# Autodesk Inventor assembly: Coluna_Suspensao_3-Cabos_Modelo3
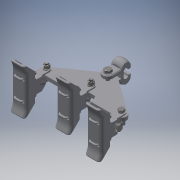
[picture p0: Inventor's stored thumbnail of the model, 180x180]
Saved by Autodesk Inventor 2018 (Build 220112000, 112)
## iProperties
Created: 2021-08-02
Part Number: Coluna_Suspensao_3-Cabos_Modelo3
Document SubType Name: Assembly
Designer: L08619
Author: L08619
## Documents named in this file (4)
- C:\Users\l08619\Documents\Projetos\TAESA\Modelo 3D - Tensionadores e Suspensão\Suporte de Suspenção\Coluna_Suspensao_3-Cabos_Modelo3.iam
- C:\Users\l08619\Documents\Projetos\TAESA\Modelo 3D - Tensionadores e Suspensão\Suporte de Suspenção\Corpo_Suporte_3_Cabos_Modelo3.ipt
- C:\Users\l08619\Documents\Projetos\TAESA\Modelo 3D - Tensionadores e Suspensão\Suporte de Suspenção\Clevis-Socket.iam
- C:\Users\l08619\Documents\Projetos\TAESA\Modelo 3D - Tensionadores e Suspensão\Suporte de Suspenção\Suspenssion_Clamp.iam
## Components (5 placed, 3 different names)
1. Corpo_Suporte_3_Cabos_Modelo3:1 — Mate:1, Mate:2, Cylindrical:1, Cylindrical:2, Cylindrical:3, Cylindrical:4
2. Clevis-Socket:1 [sub-assembly] — Cylindrical:1
3. Suspenssion_Clamp:1 [sub-assembly] — Cylindrical:2
4. Suspenssion_Clamp:2 [sub-assembly] — Cylindrical:3
5. Suspenssion_Clamp:3 [sub-assembly] — Cylindrical:4
## Relationships (6: CylindricalJoint 4, Mate 2)
- Mate:1: Corpo_Suporte_3_Cabos_Modelo3:1
- Mate:2: Corpo_Suporte_3_Cabos_Modelo3:1
- Cylindrical:1: Corpo_Suporte_3_Cabos_Modelo3:1 ↔ Clevis-Socket:1
- Cylindrical:2: Corpo_Suporte_3_Cabos_Modelo3:1 ↔ Suspenssion_Clamp:1
- Cylindrical:3: Corpo_Suporte_3_Cabos_Modelo3:1 ↔ Suspenssion_Clamp:2
- Cylindrical:4: Corpo_Suporte_3_Cabos_Modelo3:1 ↔ Suspenssion_Clamp:3
